# Autodesk Inventor assembly: Pneumatic Cylinder (double acting).ipt
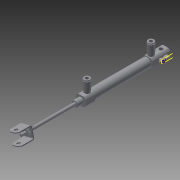
[picture p0: Inventor's stored thumbnail of the model, 180x180]
Saved by Autodesk Inventor 2015 SP1 (Build 190203100, 203)
## iProperties
Created: 2014-05-24
Part Number: Pneumatic Cylinder (double acting).ipt
Document SubType Name: Assembly
Designer: Christopher
Author: Christopher
## Documents named in this file (4)
- F:\VEX CAD Library\Motion\Pneumatic Cylinder (double acting).iam
- F:\VEX CAD Library\Motion\Pneumatic Cylinder.ipt
- F:\VEX CAD Library\Motion\pneumatic rod.ipt
- F:\VEX CAD Library\Motion\Pneumatic Bracket.ipt
## Components (3 placed, 3 different names)
1. Pneumatic Cylinder:1 — Mate:1, Mate:2, Mate:3
2. pneumatic rod:1 — Mate:1, Mate:2, Mate:3, Mate:4, Mate:5
3. Pneumatic Bracket:1 — Mate:4, Mate:5
## Relationships (5: Mate 5)
- Mate:1: Pneumatic Cylinder:1 ↔ pneumatic rod:1
- Mate:2: Pneumatic Cylinder:1 ↔ pneumatic rod:1
- Mate:3: Pneumatic Cylinder:1 ↔ pneumatic rod:1
- Mate:4: pneumatic rod:1 ↔ Pneumatic Bracket:1
- Mate:5: pneumatic rod:1 ↔ Pneumatic Bracket:1
